# Autodesk Inventor assembly: rowing_steering
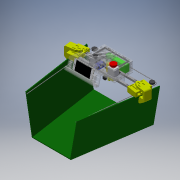
[picture p0: Inventor's stored thumbnail of the model, 180x180]
Saved by Autodesk Inventor 2019 (Build 230136000, 136)
## iProperties
Created: 2019-01-31
Part Number: rowing_steering
Document SubType Name: Assembly
Designer: suchanek
Author: suchanek
## Documents named in this file (37)
- D:\suchanek\programming\rowing_steering\model\rowing_steering.iam
- D:\suchanek\programming\rowing_steering\model\boat_segment.ipt
- D:\suchanek\programming\rowing_steering\model\holder_inner.ipt
- D:\suchanek\programming\rowing_steering\model\holder_bar.ipt
- D:\suchanek\programming\rowing_steering\model\case_base.ipt
- D:\suchanek\programming\rowing_steering\model\holder_outer.ipt
- D:\suchanek\programming\rowing_steering\model\case_back.ipt
- D:\suchanek\programming\rowing_steering\model\case_front.ipt
- D:\suchanek\programming\rowing_steering\model\case_side.ipt
- D:\suchanek\programming\rowing_steering\model\case_top.ipt
- D:\suchanek\programming\rowing_steering\model\servo.ipt
- D:\suchanek\programming\rowing_steering\model\servo_piece.ipt
- D:\suchanek\programming\rowing_steering\model\arm.ipt
- D:\suchanek\programming\rowing_steering\model\arduino-uno.snapshot.3\arduino uno.iam
- D:\suchanek\programming\rowing_steering\model\battery.ipt
- D:\suchanek\programming\rowing_steering\model\case_top_cover_slot.ipt
- D:\suchanek\programming\rowing_steering\model\bar_protector.ipt
- D:\suchanek\programming\rowing_steering\model\emergency_stop.ipt
- D:\suchanek\programming\rowing_steering\model\switch.ipt
- D:\suchanek\programming\rowing_steering\model\case_top_cover_sheet.ipt
- D:\suchanek\programming\rowing_steering\model\case_lid.ipt
- D:\suchanek\programming\rowing_steering\model\hinge.ipt
- D:\suchanek\programming\rowing_steering\model\usb_cover.ipt
- D:\suchanek\programming\rowing_steering\model\latch.ipt
- D:\suchanek\programming\rowing_steering\model\phone_holder_slider_insert.ipt
- D:\suchanek\programming\rowing_steering\model\phone_holder_slider_cover.ipt
- D:\suchanek\programming\rowing_steering\model\phone_holder_slider.ipt
- D:\suchanek\programming\rowing_steering\model\phone_holder_slider_side.ipt
- D:\suchanek\programming\rowing_steering\model\phone_holder_back.ipt
- D:\suchanek\programming\rowing_steering\model\iphone.ipt
- D:\suchanek\programming\rowing_steering\model\arm_safe.ipt
- D:\suchanek\programming\rowing_steering\model\phone_holder_botom_insert.ipt
- D:\suchanek\programming\rowing_steering\model\phone_holder_side_insert.ipt
- D:\suchanek\programming\rowing_steering\model\phone_holder_top_insert.ipt
- D:\suchanek\programming\rowing_steering\model\phone_holder_botom_cap.ipt
- D:\suchanek\programming\rowing_steering\model\phone_holder_side_cap.ipt
- D:\suchanek\programming\rowing_steering\model\phone_holder_top_cap.ipt
## Components (51 placed, 36 different names)
1. boat_segment:1 — Angle:1, Mate:44, Mate:45, Mate:47, Mate:48, Flush:8, Flush:9, Tangent:9, Angle:10, Flush:15
2. holder_inner:1 — Mate:44, Mate:45, Mate:46, Tangent:54, Symmetry:7, Angle:9, Tangent:52, Mate:52, Mate:53, Tangent:53
3. holder_inner:2 — Mate:47, Mate:48, Symmetry:7
4. holder_bar:1 — Angle:2, Mate:13, Angle:5, Tangent:6, Tangent:8, Tangent:52, Flush:8, Mate:53
5. holder_bar:2 — Angle:1, Angle:2, Tangent:7, Flush:9, Mate:52, Tangent:53
6. case_base:1 — Mate:13, Angle:5, Tangent:6, Tangent:7, Tangent:8, Mate:54, Mate:55, Flush:10, Mate:56, Mate:57, Flush:11, Mate:58, Flush:13, Mate:60, Flush:14, Mate:64, Mate:70, Mate:71, Mate:72, Mate:73, Mate:74
7. holder_outer:1 — Symmetry:4, Symmetry:5, Symmetry:6, Mate:46, Tangent:54, Angle:9, Tangent:9
8. holder_outer:2 — Symmetry:4, Symmetry:5, Symmetry:6
9. case_back:1 — Mate:56, Mate:57, Flush:11, Flush:12, Mate:59, Mate:75, Flush:16, Mate:78
10. case_front:1 — Mate:54, Mate:55, Flush:10, Mate:61, Mate:63, Angle:12, Rigid:4, Angle:13, Angle:14
11. case_side:1 — Mate:59, Mate:60, Flush:14, Mate:62, Mate:77
12. case_top:1 — Mate:61, Mate:62, Mate:63, Rigid:2, Rotational:2, Rotational:3, Flush:17, Mate:85, Mate:86, Mate:87, Mate:88, Angle:15
13. case_side:2 — Mate:58, Flush:12, Flush:13, Angle:11
14. servo:1 — Mate:64, Rotational:1, Mate:73, Mate:74
15. servo_piece:1 — Rotational:1, Mate:67, Mate:68, Mate:69, Rigid:7
16. arm:1 — Mate:67, Mate:68, Mate:69, Angle:10, Flush:15, Rigid:1
17. arduino uno:1 [sub-assembly] — Mate:70, Mate:71, Angle:11
18. battery:1 — Mate:72, Mate:75
19. case_top_cover_slot:1 — Mate:77, Rigid:3
20. bar_protector:1 — Rigid:1
21. emergency_stop:1 — Rotational:2, Angle:12
22. switch:1 — Rigid:2
23. case_top_cover_sheet:1 — Rigid:3, Flush:16, Mate:78
24. case_lid:1 — Rotational:3, Mate:79, Mate:80, Flush:18, Flush:19, Mate:82, Mate:83, Flush:22
25. hinge:1 — Mate:79, Mate:81, Flush:19, Flush:21
26. hinge:2 — Mate:80, Mate:81, Flush:17, Flush:18, Flush:20
27. usb_cover:1 — Rigid:4
28. latch:1 — Mate:83, Flush:21, Mate:84
29. phone_holder_slider_insert:1 — Mate:87, Mate:88, Angle:14, Rigid:6
30. latch:2 — Mate:82, Flush:20, Mate:84, Flush:22
31. phone_holder_slider_insert:2 — Mate:85, Mate:86, Angle:13, Rigid:5, Cylindrical:1
32. phone_holder_slider_cover:1 — Rigid:5
33. phone_holder_slider_cover:2 — Rigid:6
34. phone_holder_slider:1 — Cylindrical:1, Angle:15, Rotational:4, Angle:16, Rotational:5
35. phone_holder_slider_side:1 — Rotational:4, Angle:16, Angle:17
36. phone_holder_slider_side:2 — Rotational:5, Angle:17, Rotational:6, Angle:18
37. phone_holder_back:1 — Rotational:6, Angle:18, Mate:89, Angle:19, Slider:1, Mate:90, Rotational:7, Mate:92, Slider:2
38. iphone:1 — Mate:89, Angle:19, Mate:91, Mate:92
39. arm_safe:1 — Rigid:7
40. phone_holder_botom_insert:1 — Rigid:10, Rigid:12
41. phone_holder_side_insert:1 — Rigid:11, Rigid:14
42. phone_holder_top_insert:1 — Rigid:9, Rigid:15
43. phone_holder_botom_insert:2 — Rotational:7, Angle:20, Mate:91, Rigid:10
44. phone_holder_side_insert:2 — Rigid:8, Rigid:13
45. phone_holder_top_insert:2 — Slider:2, Rigid:9
46. phone_holder_side_insert:3 — Symmetry:8, Symmetry:9, Mate:90, Angle:20, Rigid:11
47. phone_holder_side_insert:4 — Slider:1, Symmetry:8, Symmetry:9, Rigid:8
48. phone_holder_botom_cap:1 — Rigid:12
49. phone_holder_side_cap:1 — Rigid:13
50. phone_holder_top_cap:1 — Rigid:15
51. phone_holder_side_cap:2 — Rigid:14
## Relationships (112: Mate 44, Angle 15, Flush 15, WeldJoint 15, Tangent 7, RevoluteJoint 7, Symmetry 6, TranslationJoint 2, CylindricalJoint 1)
- Angle:1 (0 deg): boat_segment:1 ↔ holder_bar:2
- Angle:2 (0 deg): holder_bar:1 ↔ holder_bar:2
- Symmetry:4: holder_outer:1 ↔ holder_outer:2
- Symmetry:5: holder_outer:1 ↔ holder_outer:2
- Symmetry:6: holder_outer:1 ↔ holder_outer:2
- Mate:13: holder_bar:1 ↔ case_base:1
- Angle:5 (0 deg): holder_bar:1 ↔ case_base:1
- Tangent:6: holder_bar:1 ↔ case_base:1
- Tangent:7: holder_bar:2 ↔ case_base:1
- Tangent:8: holder_bar:1 ↔ case_base:1
- Mate:44: boat_segment:1 ↔ holder_inner:1
- Mate:45: boat_segment:1 ↔ holder_inner:1
- Mate:46: holder_inner:1 ↔ holder_outer:1
- Mate:47: boat_segment:1 ↔ holder_inner:2
- Mate:48: boat_segment:1 ↔ holder_inner:2
- Tangent:54: holder_inner:1 ↔ holder_outer:1
- Symmetry:7: holder_inner:1 ↔ holder_inner:2
- Angle:9 (0 deg): holder_inner:1 ↔ holder_outer:1
- Tangent:52: holder_inner:1 ↔ holder_bar:1
- Flush:8: boat_segment:1 ↔ holder_bar:1
- Flush:9: boat_segment:1 ↔ holder_bar:2
- Mate:52: holder_inner:1 ↔ holder_bar:2
- Mate:53: holder_inner:1 ↔ holder_bar:1
- Tangent:9: boat_segment:1 ↔ holder_outer:1
- Tangent:53: holder_inner:1 ↔ holder_bar:2
- Mate:54: case_base:1 ↔ case_front:1
- Mate:55: case_base:1 ↔ case_front:1
- Flush:10: case_base:1 ↔ case_front:1
- Mate:56: case_base:1 ↔ case_back:1
- Mate:57: case_base:1 ↔ case_back:1
- Flush:11: case_base:1 ↔ case_back:1
- Mate:58: case_base:1 ↔ case_side:2
- Flush:12: case_back:1 ↔ case_side:2
- Flush:13: case_base:1 ↔ case_side:2
- Mate:59: case_back:1 ↔ case_side:1
- Mate:60: case_base:1 ↔ case_side:1
- Flush:14: case_base:1 ↔ case_side:1
- Mate:61: case_front:1 ↔ case_top:1
- Mate:62: case_side:1 ↔ case_top:1
- Mate:63: case_front:1 ↔ case_top:1
- Mate:64: case_base:1 ↔ servo:1
- Rotational:1 [RevoluteJoint]: servo:1 ↔ servo_piece:1
- Mate:67: servo_piece:1 ↔ arm:1
- Mate:68: servo_piece:1 ↔ arm:1
- Mate:69: servo_piece:1 ↔ arm:1
- Angle:10 (0 deg): boat_segment:1 ↔ arm:1
- Flush:15 (-37 mm): boat_segment:1 ↔ arm:1
- Mate:70 (5 mm): case_base:1 ↔ arduino uno:1
- Mate:71: case_base:1 ↔ arduino uno:1
- Angle:11 (0 deg): case_side:2 ↔ arduino uno:1
- Mate:72: case_base:1 ↔ battery:1
- Mate:73: case_base:1 ↔ servo:1
- Mate:74: case_base:1 ↔ servo:1
- Mate:75 (3 mm): case_back:1 ↔ battery:1
- Mate:77 (5 mm): case_side:1 ↔ case_top_cover_slot:1
- Rigid:1 [WeldJoint]: arm:1 ↔ bar_protector:1
- Rigid:2 [WeldJoint]: case_top:1 ↔ switch:1
- Rotational:2 [RevoluteJoint]: case_top:1 ↔ emergency_stop:1
- Angle:12 (0 deg): case_front:1 ↔ emergency_stop:1
- Rigid:3 [WeldJoint]: case_top_cover_slot:1 ↔ case_top_cover_sheet:1
- Flush:16: case_back:1 ↔ case_top_cover_sheet:1
- Mate:78: case_back:1 ↔ case_top_cover_sheet:1
- Rotational:3 [RevoluteJoint]: case_top:1 ↔ case_lid:1
- Mate:79: case_lid:1 ↔ hinge:1
- Mate:80: case_lid:1 ↔ hinge:2
- Mate:81: hinge:1 ↔ hinge:2
- Flush:17 (8.5 mm): case_top:1 ↔ hinge:2
- Flush:18 (-20 mm): case_lid:1 ↔ hinge:2
- Flush:19 (20 mm): case_lid:1 ↔ hinge:1
- Rigid:4 [WeldJoint]: case_front:1 ↔ usb_cover:1
- Mate:82: case_lid:1 ↔ latch:2
- Flush:20: hinge:2 ↔ latch:2
- Mate:83: case_lid:1 ↔ latch:1
- Flush:21: hinge:1 ↔ latch:1
- Mate:84: latch:1 ↔ latch:2
- Flush:22 (-8 mm): case_lid:1 ↔ latch:2
- Mate:85: case_top:1 ↔ phone_holder_slider_insert:2
- Mate:86: case_top:1 ↔ phone_holder_slider_insert:2
- Angle:13 (0 deg): case_front:1 ↔ phone_holder_slider_insert:2
- Mate:87: case_top:1 ↔ phone_holder_slider_insert:1
- Mate:88: case_top:1 ↔ phone_holder_slider_insert:1
- Angle:14 (0 deg): case_front:1 ↔ phone_holder_slider_insert:1
- Rigid:5 [WeldJoint]: phone_holder_slider_insert:2 ↔ phone_holder_slider_cover:1
- Rigid:6 [WeldJoint]: phone_holder_slider_insert:1 ↔ phone_holder_slider_cover:2
- Cylindrical:1: phone_holder_slider_insert:2 ↔ phone_holder_slider:1
- Angle:15 (0 deg): case_top:1 ↔ phone_holder_slider:1
- Rotational:4 [RevoluteJoint]: phone_holder_slider:1 ↔ phone_holder_slider_side:1
- Angle:16 (0 deg): phone_holder_slider:1 ↔ phone_holder_slider_side:1
- Rotational:5 [RevoluteJoint]: phone_holder_slider:1 ↔ phone_holder_slider_side:2
- Angle:17 (0 deg): phone_holder_slider_side:1 ↔ phone_holder_slider_side:2
- Rotational:6 [RevoluteJoint]: phone_holder_slider_side:2 ↔ phone_holder_back:1
- Angle:18 (0 deg): phone_holder_slider_side:2 ↔ phone_holder_back:1
- Mate:89: phone_holder_back:1 ↔ iphone:1
- Angle:19 (0 deg): phone_holder_back:1 ↔ iphone:1
- Rigid:7 [WeldJoint]: servo_piece:1 ↔ arm_safe:1
- Slider:1 [TranslationJoint]: phone_holder_back:1 ↔ phone_holder_side_insert:4
- Symmetry:8: phone_holder_side_insert:3 ↔ phone_holder_side_insert:4
- Symmetry:9: phone_holder_side_insert:3 ↔ phone_holder_side_insert:4
- Mate:90: phone_holder_back:1 ↔ phone_holder_side_insert:3
- Rotational:7 [RevoluteJoint]: phone_holder_back:1 ↔ phone_holder_botom_insert:2
- Angle:20 (0 deg): phone_holder_botom_insert:2 ↔ phone_holder_side_insert:3
- Mate:91: iphone:1 ↔ phone_holder_botom_insert:2
- Mate:92 (69 mm): phone_holder_back:1 ↔ iphone:1
- Slider:2 [TranslationJoint]: phone_holder_back:1 ↔ phone_holder_top_insert:2
- Rigid:8 [WeldJoint]: phone_holder_side_insert:2 ↔ phone_holder_side_insert:4
- Rigid:9 [WeldJoint]: phone_holder_top_insert:1 ↔ phone_holder_top_insert:2
- Rigid:10 [WeldJoint]: phone_holder_botom_insert:1 ↔ phone_holder_botom_insert:2
- Rigid:11 [WeldJoint]: phone_holder_side_insert:1 ↔ phone_holder_side_insert:3
- Rigid:12 [WeldJoint]: phone_holder_botom_insert:1 ↔ phone_holder_botom_cap:1
- Rigid:13 [WeldJoint]: phone_holder_side_insert:2 ↔ phone_holder_side_cap:1
- Rigid:14 [WeldJoint]: phone_holder_side_insert:1 ↔ phone_holder_side_cap:2
- Rigid:15 [WeldJoint]: phone_holder_top_insert:1 ↔ phone_holder_top_cap:1
